# Autodesk Inventor assembly: Antenna_unit_MIR
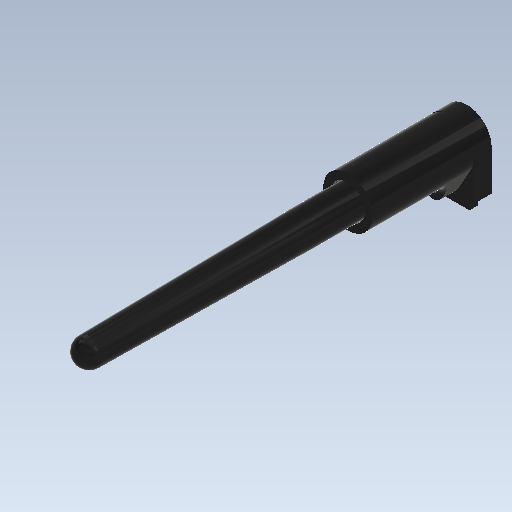
[picture p0: Inventor's stored thumbnail of the model, 512x512]
Saved by Autodesk Inventor 2020 (Build 240168000, 168)
## iProperties
Created: 2021-06-17
Part Number: Antenna_unit_MIR
Document SubType Name: Assembly
Designer: Masato Kubotera
Mass: 11.8411 g
Surface Area: 44.2768 cm^2
Volume: 8.30955 cm^3
Density: 1.425 g/cm^3
Author: Masato Kubotera
Title: Antenna_unit_MIR
## Documents named in this file (4)
- C:\Users\Masato\Documents\Inventor\CIT Brains_Inventor\OpenPlatform_ver3_0\上半身\Cockpit\Antenna_unit_MIR.iam
- C:\Users\Masato\Documents\Inventor\CIT Brains_Inventor\OpenPlatform_ver3_0\上半身\Cockpit\Antenna_frame_01_MIR.ipt
- C:\Users\Masato\Documents\Inventor\CIT Brains_Inventor\OpenPlatform_ver3_0\上半身\Cockpit\antenna.ipt
- C:\Users\Masato\Documents\Inventor\CIT Brains_Inventor\OpenPlatform_ver3_0\上半身\Cockpit\Antenna_cover_01.ipt
## Components (3 placed, 3 different names)
1. Antenna_frame_01_MIR:1 — 挿入:1, 挿入:3, 挿入:2
2. antenna:1 — 挿入:1
3. Antenna_cover_01:1 — 挿入:3, 挿入:2
## Relationships (3: Insert 3)
- 挿入:1 [Insert]: Antenna_frame_01_MIR:1 ↔ antenna:1
- 挿入:3 [Insert]: Antenna_frame_01_MIR:1 ↔ Antenna_cover_01:1
- 挿入:2 [Insert]: Antenna_frame_01_MIR:1 ↔ Antenna_cover_01:1
